# Autodesk Inventor assembly: Satellite Droit
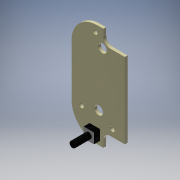
[picture p0: Inventor's stored thumbnail of the model, 180x180]
Saved by Autodesk Inventor 2019 (Build 230136000, 136)
## iProperties
Created: 2018-06-08
Part Number: Satellite Droit
Material: Générique
Document SubType Name: Assembly
Designer: dimercur
Author: dimercur
## Documents named in this file (3)
- D:\Users\dimercur\Documents locaux\Travail\git\arm-ada-ng\hardware\Box\Satellite Droit.iam
- D:\Users\dimercur\Documents locaux\Travail\git\arm-ada-ng\hardware\Box\PCB Droit.ipt
- D:\Users\dimercur\Documents locaux\Travail\git\arm-ada-ng\hardware\Box\Touch Button High.ipt
## Components (2 placed, 2 different names)
1. PCB Droit:1 — Placage:13, Placage:14, Placage:15
2. Touch Button High:1 — Placage:13, Placage:14, Placage:15
## Relationships (3: Mate 3)
- Placage:13 [Mate]: PCB Droit:1 ↔ Touch Button High:1
- Placage:14 [Mate] (2.5 mm): PCB Droit:1 ↔ Touch Button High:1
- Placage:15 [Mate] (2 mm): PCB Droit:1 ↔ Touch Button High:1
